# Autodesk Inventor assembly: GP5-100-TAV
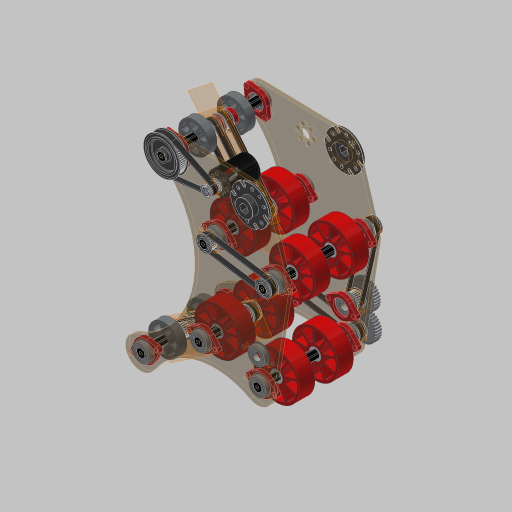
[picture p0: Inventor's stored thumbnail of the model, 512x512]
Saved by Autodesk Inventor 2023.5 (Build 275446000, 446)
## iProperties
Created: 2025-02-03
Part Number: GP5-100-TAV
Document SubType Name: Assembly
Designer: slick
Author: slick
## Documents named in this file (23)
- C:\Users\slick\OneDrive\Desktop\2025-ReefScape---CAD\Gripper\GP5\GP5-100-TAV.iam
- C:\Users\slick\OneDrive\Desktop\2025-ReefScape---CAD\Gripper\GP5\GP5-003.ipt
- C:\Users\slick\OneDrive\Desktop\2025-ReefScape---CAD\COMMON PARTS\BEARINGS\13_75mm_1_2_ThunderHex_ID_x_1_125_OD_x_0_313_WD_Flanged_Bearing_217-4006_MIR.ipt
- C:\Users\slick\OneDrive\Desktop\2025-ReefScape---CAD\Gripper\GP5\GP5-005.ipt
- C:\Users\slick\OneDrive\Desktop\2025-ReefScape---CAD\COMMON PARTS\WHEELS\2_OD_Straight_Flex_Wheel_217-6354.ipt
- C:\Users\slick\OneDrive\Desktop\2025-ReefScape---CAD\COMMON PARTS\WHEELS\am-3946 3IN 375Hex Compliant Wheel REV 3.ipt
- C:\Users\slick\OneDrive\Desktop\2025-ReefScape---CAD\COMMON PARTS\MOTORS\Minion.ipt
- C:\Users\slick\OneDrive\Desktop\2025-ReefScape---CAD\COMMON PARTS\PULLEYS\gt2\16T Gt2 Kracken PullyWCP-1178.ipt
- C:\Users\slick\OneDrive\Desktop\2025-ReefScape---CAD\COMMON PARTS\PULLEYS\gt2\60t_x_9mm_Wide_Double_Flange_Aluminum_Pulley_GT2_3mm_1_2_Hex_Bore_217-5876.ipt
- C:\Users\slick\OneDrive\Desktop\2025-ReefScape---CAD\COMMON PARTS\PULLEYS\gt2\24t_x_9mm_Wide_Double_Flange_Aluminum_Pulley_GT2_3mm_1_2_Hex_Bore_217-5875.ipt
- C:\Users\slick\OneDrive\Desktop\2025-ReefScape---CAD\COMMON PARTS\GEARS\20dp .5 hex\34t_Aluminum_Spur_Gear_20_DP_1_2_Hex_Bore_217-2706.ipt
- C:\Users\slick\OneDrive\Desktop\2025-ReefScape---CAD\Gripper\GP5\GP5-007.ipt
- C:\Users\slick\OneDrive\Desktop\2025-ReefScape---CAD\COMMON PARTS\BEARINGS\Bearing Retainer\Retainer.ipt
- C:\Users\slick\OneDrive\Desktop\2025-ReefScape---CAD\Gripper\GP5\GT2-100T.ipt
- C:\Users\slick\OneDrive\Desktop\2025-ReefScape---CAD\Gripper\GP5\GT2-90T.ipt
- C:\Users\slick\OneDrive\Desktop\2025-ReefScape---CAD\Gripper\GP5\GT2-90T16-60.ipt
- C:\Users\slick\OneDrive\Desktop\2025-ReefScape---CAD\Gripper\GP5\GT2-105T.ipt
- C:\Users\slick\OneDrive\Desktop\2025-ReefScape---CAD\Gripper\GP5\GP5-014.ipt
- C:\Users\slick\OneDrive\Desktop\2025-ReefScape---CAD\Gripper\GP5\GP5-019.ipt
- C:\Users\slick\OneDrive\Desktop\2025-ReefScape---CAD\COMMON PARTS\HUBS\WCP-1388.ipt
- C:\Users\slick\OneDrive\Desktop\2025-ReefScape---CAD\Gripper\GP5\GP5-023.ipt
- C:\Users\slick\OneDrive\Desktop\2025-ReefScape---CAD\Gripper\GP5\GP5-024.ipt
- C:\Users\slick\OneDrive\Desktop\2025-ReefScape---CAD\Gripper\GP5\GP5-025.ipt
## Components (80 placed, 22 different names)
1. Minion:1 — Mate:18, Insert:15, Mate:19, Flush:1, Mate:22
2. 34t_Aluminum_Spur_Gear_20_DP_1_2_Hex_Bore_217-2706:1 — Mate:53, Flush:16, Mate:55
3. 34t_Aluminum_Spur_Gear_20_DP_1_2_Hex_Bore_217-2706:2 — Mate:51, Flush:16, Flush:18, Mate:56, Mate:72
4. WCP-1388:1 — Mate:80, Mate:81, Insert:42
5. WCP-1388:2 — Mate:79, Mate:81, Insert:43
6. Retainer:13 — Insert:24, Insert:25
7. Retainer:12 — Insert:26, Insert:27
8. Retainer:11 — Insert:34, Insert:35
9. Retainer:10 — Insert:28, Insert:29
10. Retainer:9 — Insert:32, Insert:33
11. Retainer:8 — Insert:30, Insert:31
12. Retainer:7 — Insert:16, Insert:17
13. Retainer:6 — Insert:21, Insert:22
14. Retainer:5 — Insert:20, Insert:23
15. Retainer:4 — Insert:36, Insert:37, Insert:39
16. Retainer:3 — Insert:18, Insert:19
17. Retainer:2 — Insert:40, Insert:41
18. Retainer:1 — Insert:38, Insert:44
19. 13_75mm_1_2_ThunderHex_ID_x_1_125_OD_x_0_313_WD_Flanged_Bearing_217-4006_MIR:6 — Insert:9, Mate:13
20. 13_75mm_1_2_ThunderHex_ID_x_1_125_OD_x_0_313_WD_Flanged_Bearing_217-4006_MIR:14 — Insert:7, Mate:16, Mate:24, Mate:75
21. 13_75mm_1_2_ThunderHex_ID_x_1_125_OD_x_0_313_WD_Flanged_Bearing_217-4006_MIR:13 — Insert:8, Mate:12, Mate:64, Mate:66, Mate:67, Mate:69, Flush:73
22. 13_75mm_1_2_ThunderHex_ID_x_1_125_OD_x_0_313_WD_Flanged_Bearing_217-4006_MIR:12 — Insert:2
23. 13_75mm_1_2_ThunderHex_ID_x_1_125_OD_x_0_313_WD_Flanged_Bearing_217-4006_MIR:11 — Insert:6, Mate:74
24. 13_75mm_1_2_ThunderHex_ID_x_1_125_OD_x_0_313_WD_Flanged_Bearing_217-4006_MIR:10 — Insert:3
25. 13_75mm_1_2_ThunderHex_ID_x_1_125_OD_x_0_313_WD_Flanged_Bearing_217-4006_MIR:9 — Insert:5
26. 13_75mm_1_2_ThunderHex_ID_x_1_125_OD_x_0_313_WD_Flanged_Bearing_217-4006_MIR:8 — Insert:4
27. 13_75mm_1_2_ThunderHex_ID_x_1_125_OD_x_0_313_WD_Flanged_Bearing_217-4006_MIR:7 — Insert:1, Mate:28
28. 13_75mm_1_2_ThunderHex_ID_x_1_125_OD_x_0_313_WD_Flanged_Bearing_217-4006_MIR:5 — Insert:11, Mate:17
29. 13_75mm_1_2_ThunderHex_ID_x_1_125_OD_x_0_313_WD_Flanged_Bearing_217-4006_MIR:4 — Insert:10, Mate:14, Mate:26
30. 13_75mm_1_2_ThunderHex_ID_x_1_125_OD_x_0_313_WD_Flanged_Bearing_217-4006_MIR:3 — Insert:12, Mate:15, Mate:20, Mate:21
31. 13_75mm_1_2_ThunderHex_ID_x_1_125_OD_x_0_313_WD_Flanged_Bearing_217-4006_MIR:2 — Insert:13, Mate:50
32. 13_75mm_1_2_ThunderHex_ID_x_1_125_OD_x_0_313_WD_Flanged_Bearing_217-4006_MIR:1 — Insert:14
33. 24t_x_9mm_Wide_Double_Flange_Aluminum_Pulley_GT2_3mm_1_2_Hex_Bore_217-5875:7 — Mate:64, Mate:65
34. 24t_x_9mm_Wide_Double_Flange_Aluminum_Pulley_GT2_3mm_1_2_Hex_Bore_217-5875:8 — Mate:46, Flush:12
35. 24t_x_9mm_Wide_Double_Flange_Aluminum_Pulley_GT2_3mm_1_2_Hex_Bore_217-5875:9 — Mate:57, Mate:58, Flush:20, Mate:71
36. 24t_x_9mm_Wide_Double_Flange_Aluminum_Pulley_GT2_3mm_1_2_Hex_Bore_217-5875:10 — Mate:47, Mate:75, Flush:69, Mate:78, Flush:71, Flush:72
37. 24t_x_9mm_Wide_Double_Flange_Aluminum_Pulley_GT2_3mm_1_2_Hex_Bore_217-5875:12 — Mate:43, Mate:44, Flush:11, Flush:65
38. 24t_x_9mm_Wide_Double_Flange_Aluminum_Pulley_GT2_3mm_1_2_Hex_Bore_217-5875:13 — Mate:31, Mate:32, Flush:9, Mate:37, Mate:38, Mate:41
39. 24t_x_9mm_Wide_Double_Flange_Aluminum_Pulley_GT2_3mm_1_2_Hex_Bore_217-5875:14 — Mate:33, Mate:34, Flush:10, Mate:39, Mate:40
40. 24t_x_9mm_Wide_Double_Flange_Aluminum_Pulley_GT2_3mm_1_2_Hex_Bore_217-5875:15 — Mate:60, Mate:62, Flush:65, Flush:66, Flush:67
41. 24t_x_9mm_Wide_Double_Flange_Aluminum_Pulley_GT2_3mm_1_2_Hex_Bore_217-5875:16 — Mate:59, Mate:61, Mate:65, Flush:68
42. GT2-90T16-60:1 — Mate:22, Mate:23, Flush:2
43. GT2-105T:1 — Mate:52, Mate:54, Flush:17
44. GT2-100T:5 — Mate:69, Mate:70, Flush:68
45. GT2-90T:2 — Mate:71, Mate:72, Mate:73
46. GT2-90T:1 — Mate:77, Mate:78, Flush:71
47. GT2-100T:3 — Mate:67, Mate:68, Flush:67
48. GT2-100T:2 — Mate:36, Flush:10, Mate:44, Flush:11
49. GT2-100T:1 — Mate:35, Flush:9, Mate:45, Flush:12
50. 16T Gt2 Kracken PullyWCP-1178:1 — Mate:19, Flush:1
51. 60t_x_9mm_Wide_Double_Flange_Aluminum_Pulley_GT2_3mm_1_2_Hex_Bore_217-5876:1 — Mate:20, Mate:21, Mate:23, Flush:2, Flush:3
52. 24t_x_9mm_Wide_Double_Flange_Aluminum_Pulley_GT2_3mm_1_2_Hex_Bore_217-5875:1 — Mate:50, Flush:15, Mate:52, Mate:53, Mate:55, Flush:19
53. 24t_x_9mm_Wide_Double_Flange_Aluminum_Pulley_GT2_3mm_1_2_Hex_Bore_217-5875:2 — Mate:66, Flush:66
54. 24t_x_9mm_Wide_Double_Flange_Aluminum_Pulley_GT2_3mm_1_2_Hex_Bore_217-5875:4 — Mate:76, Mate:77, Flush:72
55. 24t_x_9mm_Wide_Double_Flange_Aluminum_Pulley_GT2_3mm_1_2_Hex_Bore_217-5875:5 — Mate:49, Flush:15, Flush:17, Mate:74, Flush:70
56. 24t_x_9mm_Wide_Double_Flange_Aluminum_Pulley_GT2_3mm_1_2_Hex_Bore_217-5875:6 — Mate:56, Flush:19, Mate:58, Mate:73
57. GP5-014:1 — Mate:32, Mate:33, Mate:35, Mate:36, Mate:38, Mate:39
58. GP5-014:2 — Mate:59, Mate:60, Mate:61, Mate:62, Mate:63
59. GP5-019:1 — Mate:31, Mate:37, Mate:42
60. GP5-019:2 — Mate:34, Mate:40
61. GP5-003:1 — Mate:1, Mate:2, Mate:3, Insert:1, Insert:2, Insert:3, Insert:4, Insert:5, Insert:6, Insert:13, Insert:16, Insert:17, Insert:18, Insert:19, Insert:20, Insert:21, Insert:22, Insert:23, Insert:36, Insert:37, Insert:38, Insert:39, Insert:40, Insert:41, Mate:80, Insert:42, Insert:44
62. GP5-003:2 — Mate:1, Mate:2, Mate:3, Insert:7, Insert:8, Insert:9, Insert:10, Insert:11, Insert:12, Insert:14, Mate:18, Insert:15, Mate:29, Insert:24, Insert:25, Insert:26, Insert:27, Insert:28, Insert:29, Insert:30, Insert:31, Insert:32, Insert:33, Insert:34, Insert:35, Mate:79, Insert:43
63. GP5-007:1 — Mate:15, Flush:3
64. GP5-025:1 — Mate:12, Mate:27, Flush:73
65. GP5-023:2 — Mate:11, Mate:13, Mate:57, Flush:20, Mate:63, Mate:68, Mate:70
66. GP5-023:1 — Mate:16, Mate:47, Flush:69
67. GP5-024:1 — Mate:14, Mate:51, Flush:18
68. GP5-005:6 — Mate:17, Mate:25, Mate:49, Mate:54, Flush:70, Mate:76
69. am-3946 3IN 375Hex Compliant Wheel REV 3:3 — Mate:26, Flush:5, Flush:6
70. am-3946 3IN 375Hex Compliant Wheel REV 3:2 — Mate:25, Flush:4, Flush:5
71. am-3946 3IN 375Hex Compliant Wheel REV 3:1 — Mate:24, Flush:4, Mate:43
72. am-3946 3IN 375Hex Compliant Wheel REV 3:4 — Mate:11, Flush:6, Flush:8, Mate:29
73. 2_OD_Straight_Flex_Wheel_217-6354:1 — Mate:28, Flush:7
74. 2_OD_Straight_Flex_Wheel_217-6354:2 — Mate:27, Flush:7, Flush:8
75. am-3946 3IN 375Hex Compliant Wheel REV 3:5
76. am-3946 3IN 375Hex Compliant Wheel REV 3:6
77. am-3946 3IN 375Hex Compliant Wheel REV 3:7 — Mate:45, Mate:46
78. am-3946 3IN 375Hex Compliant Wheel REV 3:8
79. 2_OD_Straight_Flex_Wheel_217-6354:3 — Mate:41, Mate:42
80. 2_OD_Straight_Flex_Wheel_217-6354:4
## Component patterns: (2 elements, first: am-3946 3IN 375Hex Compliant Wheel REV 3:3 + am-3946 3IN 375Hex Compliant Wheel REV 3:2 + am-3946 3IN 375Hex Compliant Wheel REV 3:1 + am-3946 3IN 375Hex Compliant Wheel REV 3:4 + 2_OD_Straight_Flex_Wheel_217-6354:1 + 2_OD_Straight_Flex_Wheel_217-6354:2)
## Relationships (143: Mate 72, Insert 44, Flush 27)
- Mate:1: GP5-003:1 ↔ GP5-003:2
- Mate:2: GP5-003:1 ↔ GP5-003:2
- Mate:3 (139.7 mm): GP5-003:1 ↔ GP5-003:2
- Mate:11: GP5-023:2 ↔ am-3946 3IN 375Hex Compliant Wheel REV 3:4
- Insert:1: 13_75mm_1_2_ThunderHex_ID_x_1_125_OD_x_0_313_WD_Flanged_Bearing_217-4006_MIR:7 ↔ GP5-003:1
- Insert:2: 13_75mm_1_2_ThunderHex_ID_x_1_125_OD_x_0_313_WD_Flanged_Bearing_217-4006_MIR:12 ↔ GP5-003:1
- Insert:3: 13_75mm_1_2_ThunderHex_ID_x_1_125_OD_x_0_313_WD_Flanged_Bearing_217-4006_MIR:10 ↔ GP5-003:1
- Insert:4: 13_75mm_1_2_ThunderHex_ID_x_1_125_OD_x_0_313_WD_Flanged_Bearing_217-4006_MIR:8 ↔ GP5-003:1
- Insert:5: 13_75mm_1_2_ThunderHex_ID_x_1_125_OD_x_0_313_WD_Flanged_Bearing_217-4006_MIR:9 ↔ GP5-003:1
- Insert:6: 13_75mm_1_2_ThunderHex_ID_x_1_125_OD_x_0_313_WD_Flanged_Bearing_217-4006_MIR:11 ↔ GP5-003:1
- Insert:7: 13_75mm_1_2_ThunderHex_ID_x_1_125_OD_x_0_313_WD_Flanged_Bearing_217-4006_MIR:14 ↔ GP5-003:2
- Insert:8: 13_75mm_1_2_ThunderHex_ID_x_1_125_OD_x_0_313_WD_Flanged_Bearing_217-4006_MIR:13 ↔ GP5-003:2
- Insert:9: 13_75mm_1_2_ThunderHex_ID_x_1_125_OD_x_0_313_WD_Flanged_Bearing_217-4006_MIR:6 ↔ GP5-003:2
- Insert:10: 13_75mm_1_2_ThunderHex_ID_x_1_125_OD_x_0_313_WD_Flanged_Bearing_217-4006_MIR:4 ↔ GP5-003:2
- Insert:11: 13_75mm_1_2_ThunderHex_ID_x_1_125_OD_x_0_313_WD_Flanged_Bearing_217-4006_MIR:5 ↔ GP5-003:2
- Insert:12: 13_75mm_1_2_ThunderHex_ID_x_1_125_OD_x_0_313_WD_Flanged_Bearing_217-4006_MIR:3 ↔ GP5-003:2
- Insert:13: 13_75mm_1_2_ThunderHex_ID_x_1_125_OD_x_0_313_WD_Flanged_Bearing_217-4006_MIR:2 ↔ GP5-003:1
- Insert:14: 13_75mm_1_2_ThunderHex_ID_x_1_125_OD_x_0_313_WD_Flanged_Bearing_217-4006_MIR:1 ↔ GP5-003:2
- Mate:12: 13_75mm_1_2_ThunderHex_ID_x_1_125_OD_x_0_313_WD_Flanged_Bearing_217-4006_MIR:13 ↔ GP5-025:1
- Mate:13: 13_75mm_1_2_ThunderHex_ID_x_1_125_OD_x_0_313_WD_Flanged_Bearing_217-4006_MIR:6 ↔ GP5-023:2
- Mate:14: 13_75mm_1_2_ThunderHex_ID_x_1_125_OD_x_0_313_WD_Flanged_Bearing_217-4006_MIR:4 ↔ GP5-024:1
- Mate:15: 13_75mm_1_2_ThunderHex_ID_x_1_125_OD_x_0_313_WD_Flanged_Bearing_217-4006_MIR:3 ↔ GP5-007:1
- Mate:16: 13_75mm_1_2_ThunderHex_ID_x_1_125_OD_x_0_313_WD_Flanged_Bearing_217-4006_MIR:14 ↔ GP5-023:1
- Mate:17: 13_75mm_1_2_ThunderHex_ID_x_1_125_OD_x_0_313_WD_Flanged_Bearing_217-4006_MIR:5 ↔ GP5-005:6
- Mate:18: Minion:1 ↔ GP5-003:2
- Insert:15: Minion:1 ↔ GP5-003:2
- Mate:19: Minion:1 ↔ 16T Gt2 Kracken PullyWCP-1178:1
- Flush:1: Minion:1 ↔ 16T Gt2 Kracken PullyWCP-1178:1
- Mate:20: 13_75mm_1_2_ThunderHex_ID_x_1_125_OD_x_0_313_WD_Flanged_Bearing_217-4006_MIR:3 ↔ 60t_x_9mm_Wide_Double_Flange_Aluminum_Pulley_GT2_3mm_1_2_Hex_Bore_217-5876:1
- Mate:21: 13_75mm_1_2_ThunderHex_ID_x_1_125_OD_x_0_313_WD_Flanged_Bearing_217-4006_MIR:3 ↔ 60t_x_9mm_Wide_Double_Flange_Aluminum_Pulley_GT2_3mm_1_2_Hex_Bore_217-5876:1
- Mate:22: Minion:1 ↔ GT2-90T16-60:1
- Mate:23 (0.0762 mm): GT2-90T16-60:1 ↔ 60t_x_9mm_Wide_Double_Flange_Aluminum_Pulley_GT2_3mm_1_2_Hex_Bore_217-5876:1
- Flush:2: GT2-90T16-60:1 ↔ 60t_x_9mm_Wide_Double_Flange_Aluminum_Pulley_GT2_3mm_1_2_Hex_Bore_217-5876:1
- Flush:3: 60t_x_9mm_Wide_Double_Flange_Aluminum_Pulley_GT2_3mm_1_2_Hex_Bore_217-5876:1 ↔ GP5-007:1
- Mate:24: 13_75mm_1_2_ThunderHex_ID_x_1_125_OD_x_0_313_WD_Flanged_Bearing_217-4006_MIR:14 ↔ am-3946 3IN 375Hex Compliant Wheel REV 3:1
- Mate:25: GP5-005:6 ↔ am-3946 3IN 375Hex Compliant Wheel REV 3:2
- Mate:26: 13_75mm_1_2_ThunderHex_ID_x_1_125_OD_x_0_313_WD_Flanged_Bearing_217-4006_MIR:4 ↔ am-3946 3IN 375Hex Compliant Wheel REV 3:3
- Flush:4: am-3946 3IN 375Hex Compliant Wheel REV 3:2 ↔ am-3946 3IN 375Hex Compliant Wheel REV 3:1
- Flush:5: am-3946 3IN 375Hex Compliant Wheel REV 3:3 ↔ am-3946 3IN 375Hex Compliant Wheel REV 3:2
- Flush:6: am-3946 3IN 375Hex Compliant Wheel REV 3:3 ↔ am-3946 3IN 375Hex Compliant Wheel REV 3:4
- Mate:27: GP5-025:1 ↔ 2_OD_Straight_Flex_Wheel_217-6354:2
- Mate:28: 13_75mm_1_2_ThunderHex_ID_x_1_125_OD_x_0_313_WD_Flanged_Bearing_217-4006_MIR:7 ↔ 2_OD_Straight_Flex_Wheel_217-6354:1
- Flush:7: 2_OD_Straight_Flex_Wheel_217-6354:1 ↔ 2_OD_Straight_Flex_Wheel_217-6354:2
- Flush:8 (6.35 mm): am-3946 3IN 375Hex Compliant Wheel REV 3:4 ↔ 2_OD_Straight_Flex_Wheel_217-6354:2
- Mate:29 (25.4 mm): GP5-003:2 ↔ am-3946 3IN 375Hex Compliant Wheel REV 3:4
- Mate:31: 24t_x_9mm_Wide_Double_Flange_Aluminum_Pulley_GT2_3mm_1_2_Hex_Bore_217-5875:13 ↔ GP5-019:1
- Mate:32: 24t_x_9mm_Wide_Double_Flange_Aluminum_Pulley_GT2_3mm_1_2_Hex_Bore_217-5875:13 ↔ GP5-014:1
- Mate:33: 24t_x_9mm_Wide_Double_Flange_Aluminum_Pulley_GT2_3mm_1_2_Hex_Bore_217-5875:14 ↔ GP5-014:1
- Mate:34: 24t_x_9mm_Wide_Double_Flange_Aluminum_Pulley_GT2_3mm_1_2_Hex_Bore_217-5875:14 ↔ GP5-019:2
- Mate:35: GT2-100T:1 ↔ GP5-014:1
- Mate:36: GT2-100T:2 ↔ GP5-014:1
- Flush:9: 24t_x_9mm_Wide_Double_Flange_Aluminum_Pulley_GT2_3mm_1_2_Hex_Bore_217-5875:13 ↔ GT2-100T:1
- Flush:10: 24t_x_9mm_Wide_Double_Flange_Aluminum_Pulley_GT2_3mm_1_2_Hex_Bore_217-5875:14 ↔ GT2-100T:2
- Mate:37: 24t_x_9mm_Wide_Double_Flange_Aluminum_Pulley_GT2_3mm_1_2_Hex_Bore_217-5875:13 ↔ GP5-019:1
- Mate:38: 24t_x_9mm_Wide_Double_Flange_Aluminum_Pulley_GT2_3mm_1_2_Hex_Bore_217-5875:13 ↔ GP5-014:1
- Mate:39: 24t_x_9mm_Wide_Double_Flange_Aluminum_Pulley_GT2_3mm_1_2_Hex_Bore_217-5875:14 ↔ GP5-014:1
- Mate:40: 24t_x_9mm_Wide_Double_Flange_Aluminum_Pulley_GT2_3mm_1_2_Hex_Bore_217-5875:14 ↔ GP5-019:2
- Mate:41: 24t_x_9mm_Wide_Double_Flange_Aluminum_Pulley_GT2_3mm_1_2_Hex_Bore_217-5875:13 ↔ 2_OD_Straight_Flex_Wheel_217-6354:3
- Mate:42: GP5-019:1 ↔ 2_OD_Straight_Flex_Wheel_217-6354:3
- Insert:16: Retainer:7 ↔ GP5-003:1
- Insert:17: Retainer:7 ↔ GP5-003:1
- Insert:18: Retainer:3 ↔ GP5-003:1
- Insert:19: Retainer:3 ↔ GP5-003:1
- Insert:20: Retainer:5 ↔ GP5-003:1
- Insert:21: Retainer:6 ↔ GP5-003:1
- Insert:22: Retainer:6 ↔ GP5-003:1
- Insert:23: Retainer:5 ↔ GP5-003:1
- Insert:24: Retainer:13 ↔ GP5-003:2
- Insert:25: Retainer:13 ↔ GP5-003:2
- Insert:26: Retainer:12 ↔ GP5-003:2
- Insert:27: Retainer:12 ↔ GP5-003:2
- Insert:28: Retainer:10 ↔ GP5-003:2
- Insert:29: Retainer:10 ↔ GP5-003:2
- Insert:30: Retainer:8 ↔ GP5-003:2
- Insert:31: Retainer:8 ↔ GP5-003:2
- Insert:32: Retainer:9 ↔ GP5-003:2
- Insert:33: Retainer:9 ↔ GP5-003:2
- Insert:34: Retainer:11 ↔ GP5-003:2
- Insert:35: Retainer:11 ↔ GP5-003:2
- Insert:36: Retainer:4 ↔ GP5-003:1
- Insert:37: Retainer:4 ↔ GP5-003:1
- Insert:38: Retainer:1 ↔ GP5-003:1
- Insert:39: Retainer:4 ↔ GP5-003:1
- Insert:40: Retainer:2 ↔ GP5-003:1
- Insert:41: Retainer:2 ↔ GP5-003:1
- Mate:43: 24t_x_9mm_Wide_Double_Flange_Aluminum_Pulley_GT2_3mm_1_2_Hex_Bore_217-5875:12 ↔ am-3946 3IN 375Hex Compliant Wheel REV 3:1
- Mate:44 (0.0762 mm): 24t_x_9mm_Wide_Double_Flange_Aluminum_Pulley_GT2_3mm_1_2_Hex_Bore_217-5875:12 ↔ GT2-100T:2
- Flush:11: 24t_x_9mm_Wide_Double_Flange_Aluminum_Pulley_GT2_3mm_1_2_Hex_Bore_217-5875:12 ↔ GT2-100T:2
- Mate:45 (0.0762 mm): GT2-100T:1 ↔ am-3946 3IN 375Hex Compliant Wheel REV 3:7
- Mate:46: 24t_x_9mm_Wide_Double_Flange_Aluminum_Pulley_GT2_3mm_1_2_Hex_Bore_217-5875:8 ↔ am-3946 3IN 375Hex Compliant Wheel REV 3:7
- Flush:12: 24t_x_9mm_Wide_Double_Flange_Aluminum_Pulley_GT2_3mm_1_2_Hex_Bore_217-5875:8 ↔ GT2-100T:1
- Mate:47: 24t_x_9mm_Wide_Double_Flange_Aluminum_Pulley_GT2_3mm_1_2_Hex_Bore_217-5875:10 ↔ GP5-023:1
- Mate:49: 24t_x_9mm_Wide_Double_Flange_Aluminum_Pulley_GT2_3mm_1_2_Hex_Bore_217-5875:5 ↔ GP5-005:6
- Mate:50: 13_75mm_1_2_ThunderHex_ID_x_1_125_OD_x_0_313_WD_Flanged_Bearing_217-4006_MIR:2 ↔ 24t_x_9mm_Wide_Double_Flange_Aluminum_Pulley_GT2_3mm_1_2_Hex_Bore_217-5875:1
- Flush:15: 24t_x_9mm_Wide_Double_Flange_Aluminum_Pulley_GT2_3mm_1_2_Hex_Bore_217-5875:1 ↔ 24t_x_9mm_Wide_Double_Flange_Aluminum_Pulley_GT2_3mm_1_2_Hex_Bore_217-5875:5
- Mate:51: 34t_Aluminum_Spur_Gear_20_DP_1_2_Hex_Bore_217-2706:2 ↔ GP5-024:1
- Mate:52: GT2-105T:1 ↔ 24t_x_9mm_Wide_Double_Flange_Aluminum_Pulley_GT2_3mm_1_2_Hex_Bore_217-5875:1
- Mate:53: 34t_Aluminum_Spur_Gear_20_DP_1_2_Hex_Bore_217-2706:1 ↔ 24t_x_9mm_Wide_Double_Flange_Aluminum_Pulley_GT2_3mm_1_2_Hex_Bore_217-5875:1
- Flush:16: 34t_Aluminum_Spur_Gear_20_DP_1_2_Hex_Bore_217-2706:1 ↔ 34t_Aluminum_Spur_Gear_20_DP_1_2_Hex_Bore_217-2706:2
- Mate:54 (0.0762 mm): GT2-105T:1 ↔ GP5-005:6
- Flush:17: GT2-105T:1 ↔ 24t_x_9mm_Wide_Double_Flange_Aluminum_Pulley_GT2_3mm_1_2_Hex_Bore_217-5875:5
- Mate:55 (1.5875 mm): 34t_Aluminum_Spur_Gear_20_DP_1_2_Hex_Bore_217-2706:1 ↔ 24t_x_9mm_Wide_Double_Flange_Aluminum_Pulley_GT2_3mm_1_2_Hex_Bore_217-5875:1
- Flush:18: 34t_Aluminum_Spur_Gear_20_DP_1_2_Hex_Bore_217-2706:2 ↔ GP5-024:1
- Mate:56: 34t_Aluminum_Spur_Gear_20_DP_1_2_Hex_Bore_217-2706:2 ↔ 24t_x_9mm_Wide_Double_Flange_Aluminum_Pulley_GT2_3mm_1_2_Hex_Bore_217-5875:6
- Flush:19: 24t_x_9mm_Wide_Double_Flange_Aluminum_Pulley_GT2_3mm_1_2_Hex_Bore_217-5875:1 ↔ 24t_x_9mm_Wide_Double_Flange_Aluminum_Pulley_GT2_3mm_1_2_Hex_Bore_217-5875:6
- Mate:57: 24t_x_9mm_Wide_Double_Flange_Aluminum_Pulley_GT2_3mm_1_2_Hex_Bore_217-5875:9 ↔ GP5-023:2
- Mate:58: 24t_x_9mm_Wide_Double_Flange_Aluminum_Pulley_GT2_3mm_1_2_Hex_Bore_217-5875:9 ↔ 24t_x_9mm_Wide_Double_Flange_Aluminum_Pulley_GT2_3mm_1_2_Hex_Bore_217-5875:6
- Flush:20: 24t_x_9mm_Wide_Double_Flange_Aluminum_Pulley_GT2_3mm_1_2_Hex_Bore_217-5875:9 ↔ GP5-023:2
- Mate:59: 24t_x_9mm_Wide_Double_Flange_Aluminum_Pulley_GT2_3mm_1_2_Hex_Bore_217-5875:16 ↔ GP5-014:2
- Mate:60: 24t_x_9mm_Wide_Double_Flange_Aluminum_Pulley_GT2_3mm_1_2_Hex_Bore_217-5875:15 ↔ GP5-014:2
- Mate:61: 24t_x_9mm_Wide_Double_Flange_Aluminum_Pulley_GT2_3mm_1_2_Hex_Bore_217-5875:16 ↔ GP5-014:2
- Mate:62: 24t_x_9mm_Wide_Double_Flange_Aluminum_Pulley_GT2_3mm_1_2_Hex_Bore_217-5875:15 ↔ GP5-014:2
- Mate:63: GP5-014:2 ↔ GP5-023:2
- Flush:65: 24t_x_9mm_Wide_Double_Flange_Aluminum_Pulley_GT2_3mm_1_2_Hex_Bore_217-5875:12 ↔ 24t_x_9mm_Wide_Double_Flange_Aluminum_Pulley_GT2_3mm_1_2_Hex_Bore_217-5875:15
- Mate:64: 13_75mm_1_2_ThunderHex_ID_x_1_125_OD_x_0_313_WD_Flanged_Bearing_217-4006_MIR:13 ↔ 24t_x_9mm_Wide_Double_Flange_Aluminum_Pulley_GT2_3mm_1_2_Hex_Bore_217-5875:7
- Mate:65: 24t_x_9mm_Wide_Double_Flange_Aluminum_Pulley_GT2_3mm_1_2_Hex_Bore_217-5875:7 ↔ 24t_x_9mm_Wide_Double_Flange_Aluminum_Pulley_GT2_3mm_1_2_Hex_Bore_217-5875:16
- Mate:66: 13_75mm_1_2_ThunderHex_ID_x_1_125_OD_x_0_313_WD_Flanged_Bearing_217-4006_MIR:13 ↔ 24t_x_9mm_Wide_Double_Flange_Aluminum_Pulley_GT2_3mm_1_2_Hex_Bore_217-5875:2
- Flush:66: 24t_x_9mm_Wide_Double_Flange_Aluminum_Pulley_GT2_3mm_1_2_Hex_Bore_217-5875:15 ↔ 24t_x_9mm_Wide_Double_Flange_Aluminum_Pulley_GT2_3mm_1_2_Hex_Bore_217-5875:2
- Mate:67: 13_75mm_1_2_ThunderHex_ID_x_1_125_OD_x_0_313_WD_Flanged_Bearing_217-4006_MIR:13 ↔ GT2-100T:3
- Mate:68 (0.0508 mm): GT2-100T:3 ↔ GP5-023:2
- Flush:67: 24t_x_9mm_Wide_Double_Flange_Aluminum_Pulley_GT2_3mm_1_2_Hex_Bore_217-5875:15 ↔ GT2-100T:3
- Mate:69: 13_75mm_1_2_ThunderHex_ID_x_1_125_OD_x_0_313_WD_Flanged_Bearing_217-4006_MIR:13 ↔ GT2-100T:5
- Mate:70 (0.0508 mm): GT2-100T:5 ↔ GP5-023:2
- Flush:68: 24t_x_9mm_Wide_Double_Flange_Aluminum_Pulley_GT2_3mm_1_2_Hex_Bore_217-5875:16 ↔ GT2-100T:5
- Mate:71: 24t_x_9mm_Wide_Double_Flange_Aluminum_Pulley_GT2_3mm_1_2_Hex_Bore_217-5875:9 ↔ GT2-90T:2
- Mate:72 (0.0508 mm): 34t_Aluminum_Spur_Gear_20_DP_1_2_Hex_Bore_217-2706:2 ↔ GT2-90T:2
- Mate:73: GT2-90T:2 ↔ 24t_x_9mm_Wide_Double_Flange_Aluminum_Pulley_GT2_3mm_1_2_Hex_Bore_217-5875:6
- Mate:74 (1.5875 mm): 13_75mm_1_2_ThunderHex_ID_x_1_125_OD_x_0_313_WD_Flanged_Bearing_217-4006_MIR:11 ↔ 24t_x_9mm_Wide_Double_Flange_Aluminum_Pulley_GT2_3mm_1_2_Hex_Bore_217-5875:5
- Mate:75 (1.5875 mm): 13_75mm_1_2_ThunderHex_ID_x_1_125_OD_x_0_313_WD_Flanged_Bearing_217-4006_MIR:14 ↔ 24t_x_9mm_Wide_Double_Flange_Aluminum_Pulley_GT2_3mm_1_2_Hex_Bore_217-5875:10
- Flush:69: 24t_x_9mm_Wide_Double_Flange_Aluminum_Pulley_GT2_3mm_1_2_Hex_Bore_217-5875:10 ↔ GP5-023:1
- Flush:70: 24t_x_9mm_Wide_Double_Flange_Aluminum_Pulley_GT2_3mm_1_2_Hex_Bore_217-5875:5 ↔ GP5-005:6
- Mate:76: 24t_x_9mm_Wide_Double_Flange_Aluminum_Pulley_GT2_3mm_1_2_Hex_Bore_217-5875:4 ↔ GP5-005:6
- Mate:77: GT2-90T:1 ↔ 24t_x_9mm_Wide_Double_Flange_Aluminum_Pulley_GT2_3mm_1_2_Hex_Bore_217-5875:4
- Mate:78 (0.0508 mm): 24t_x_9mm_Wide_Double_Flange_Aluminum_Pulley_GT2_3mm_1_2_Hex_Bore_217-5875:10 ↔ GT2-90T:1
- Flush:71: 24t_x_9mm_Wide_Double_Flange_Aluminum_Pulley_GT2_3mm_1_2_Hex_Bore_217-5875:10 ↔ GT2-90T:1
- Flush:72: 24t_x_9mm_Wide_Double_Flange_Aluminum_Pulley_GT2_3mm_1_2_Hex_Bore_217-5875:10 ↔ 24t_x_9mm_Wide_Double_Flange_Aluminum_Pulley_GT2_3mm_1_2_Hex_Bore_217-5875:4
- Flush:73: 13_75mm_1_2_ThunderHex_ID_x_1_125_OD_x_0_313_WD_Flanged_Bearing_217-4006_MIR:13 ↔ GP5-025:1
- Mate:79: WCP-1388:2 ↔ GP5-003:2
- Mate:80: WCP-1388:1 ↔ GP5-003:1
- Mate:81: WCP-1388:1 ↔ WCP-1388:2
- Insert:42: WCP-1388:1 ↔ GP5-003:1
- Insert:43: WCP-1388:2 ↔ GP5-003:2
- Insert:44: Retainer:1 ↔ GP5-003:1
